# Autodesk Inventor assembly: 2.0 Flex Wheel with insert
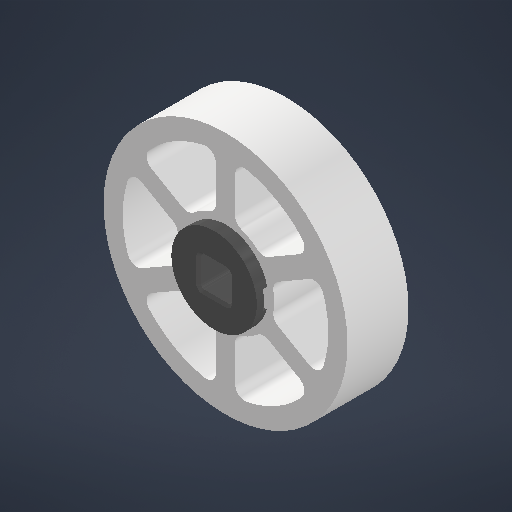
[picture p0: Inventor's stored thumbnail of the model, 512x512]
Saved by Autodesk Inventor 2025 (Build 290162000, 162)
## iProperties
Created: 2024-12-14
Part Number: 2.0 Flex Wheel with insert
Document SubType Name: Assembly
Designer: Juan
Author: Juan
## Documents named in this file (4)
- C:\Users\Juan\Documents\GitHub\ATUM-VRC-High-Stakes-CAD\Protobot\2.0 Flex Wheel with insert.iam
- C:\Users\Juan\Documents\GitHub\ATUM-VRC-High-Stakes-CAD\VEX-CAD-Inventor\Motion\Wheels\Flex Wheels\2.000 Flex Wheel\2.000 30A .500.ipt
- C:\Users\Juan\Documents\GitHub\ATUM-VRC-High-Stakes-CAD\VEX-CAD-Inventor\Motion\Wheels\Flex Wheels\2.000 Flex Wheel.ipt
- C:\Users\Juan\Documents\GitHub\ATUM-VRC-High-Stakes-CAD\VEX-CAD-Inventor\Motion\Wheels\Flex Wheels\VersaHex Adapters .250.ipt
## Components (3 placed, 2 different names)
1. 2.000 30A .500:1 — Mate:1, Mate:2, Mate:3, Mate:4
2. VersaHex Adapters .250:1 — Mate:2, Flush:1, Mate:3
3. VersaHex Adapters .250:2 — Mate:1, Flush:1, Mate:4
## Relationships (5: Mate 4, Flush 1)
- Mate:1: 2.000 30A .500:1 ↔ VersaHex Adapters .250:2
- Mate:2: 2.000 30A .500:1 ↔ VersaHex Adapters .250:1
- Flush:1: VersaHex Adapters .250:1 ↔ VersaHex Adapters .250:2
- Mate:3: 2.000 30A .500:1 ↔ VersaHex Adapters .250:1
- Mate:4: 2.000 30A .500:1 ↔ VersaHex Adapters .250:2
